# Autodesk Inventor assembly: Kepala
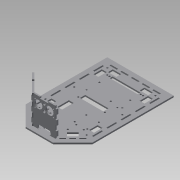
[picture p0: Inventor's stored thumbnail of the model, 180x180]
Saved by Autodesk Inventor 2015 SP1 (Build 190203100, 203)
## iProperties
Created: 2015-02-15
Part Number: Kepala
Document SubType Name: Assembly
Designer: Rafi Kurnia Putra
Author: Rafi Kurnia Putra
## Documents named in this file (4)
- D:\Dropbox\krpai berkaki trui 2015\ROBUSTA\MEKANIK\ROBUSTA\Laser Cutting\V2\Kepala.iam
- D:\Dropbox\krpai berkaki trui 2015\ROBUSTA\MEKANIK\ROBUSTA\Laser Cutting\V2\base kepala.ipt
- D:\Dropbox\krpai berkaki trui 2015\ROBUSTA\MEKANIK\ROBUSTA\Laser Cutting\V2\srf depan.ipt
- D:\Dropbox\krpai berkaki trui 2015\ROBUSTA\MEKANIK\ROBUSTA\Laser Cutting\V2\srf diag kanan.ipt
## Components (3 placed, 3 different names)
1. base kepala:1 — Flush:1, Flush:2, Flush:3, Mate:1, Mate:2, Mate:3, Mate:4, Mate:5, Mate:6
2. srf depan:1 — Mate:1, Mate:2, Mate:3
3. srf diag kanan:1 — Mate:4, Mate:5, Mate:6
## Relationships (9: Mate 6, Flush 3)
- Flush:1: base kepala:1
- Flush:2: base kepala:1
- Flush:3: base kepala:1
- Mate:1: base kepala:1 ↔ srf depan:1
- Mate:2: base kepala:1 ↔ srf depan:1
- Mate:3: base kepala:1 ↔ srf depan:1
- Mate:4: base kepala:1 ↔ srf diag kanan:1
- Mate:5: base kepala:1 ↔ srf diag kanan:1
- Mate:6: base kepala:1 ↔ srf diag kanan:1
